# Autodesk Inventor assembly: N20withBracket
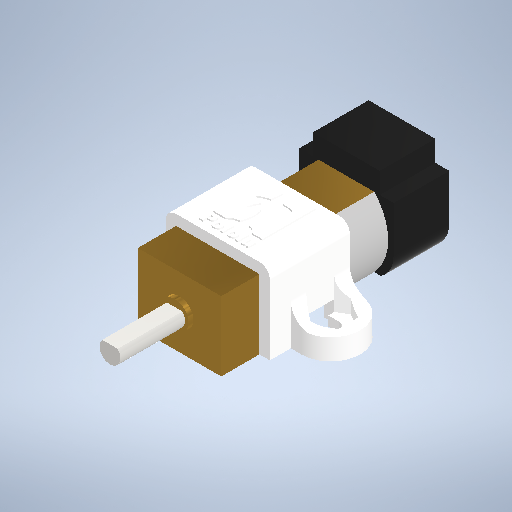
[picture p0: Inventor's stored thumbnail of the model, 512x512]
Saved by Autodesk Inventor 2025.3 (Build 293356000, 356)
## iProperties
Created: 2025-05-26
Part Number: N20withBracket
Document SubType Name: Assembly
Designer: yamashita1
Author: yamashita1
## Documents named in this file (3)
- G:\マイドライブ\project\micro-mouse\3D-Model\N20withBracket.iam
- G:\マイドライブ\project\micro-mouse\3D-Model\MercuryN20.ipt
- G:\マイドライブ\project\micro-mouse\3D-Model\micro-metal-gearmotor-bracket.ipt
## Components (2 placed, 2 different names)
1. MercuryN20:1 — メイト:1, メイト:2, フラッシュ:1
2. micro-metal-gearmotor-bracket:1 — メイト:1, メイト:2, フラッシュ:1
## Relationships (3: Mate 2, Flush 1)
- メイト:1 [Mate]: MercuryN20:1 ↔ micro-metal-gearmotor-bracket:1
- メイト:2 [Mate]: MercuryN20:1 ↔ micro-metal-gearmotor-bracket:1
- フラッシュ:1 [Flush] (5.5 mm): MercuryN20:1 ↔ micro-metal-gearmotor-bracket:1
